# Autodesk Inventor assembly: ПД Модуль 200х140х75
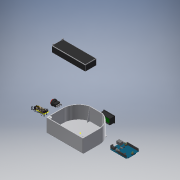
[picture p0: Inventor's stored thumbnail of the model, 180x180]
Saved by Autodesk Inventor 2019 (Build 230136000, 136)
## iProperties
Created: 2020-05-19
Part Number: ПД Модуль 200х140х75
Material: Типовые
Document SubType Name: Assembly
Designer: Surflay
Author: Surflay
## Documents named in this file (9)
- C:\Users\bossl\Desktop\Модуль ДУ Inventor\Дистанционная связь (модуль)\ПД Модуль 160х140х75.iam
- C:\Users\bossl\Desktop\Модуль ДУ Inventor\Дистанционная связь (модуль)\ПД Коробка 160х140х75.ipt
- C:\Users\bossl\Desktop\Модуль ДУ Inventor\Дистанционная связь (модуль)\РадиоМодуль.ipt
- C:\Users\bossl\Desktop\Модуль ДУ Inventor\Дистанционная связь (модуль)\Arduino UNO.ipt
- C:\Users\bossl\Desktop\Модуль ДУ Inventor\Дистанционная связь (модуль)\Аккумулятор.ipt
- C:\Users\bossl\Desktop\Модуль ДУ Inventor\Дистанционная связь (модуль)\Кнопка.ipt
- C:\Users\bossl\Desktop\Модуль ДУ Inventor\Дистанционная связь (модуль)\ВольтметрЦифровой.ipt
- C:\Users\bossl\Desktop\Модуль ДУ Inventor\Дистанционная связь (модуль)\NextionDisplay.ipt
- C:\Users\bossl\Desktop\Модуль ДУ Inventor\Дистанционная связь (модуль)\Джойстик.ipt
## Components (9 placed, 8 different names)
1. ПД Коробка 160х140х75:1
2. РадиоМодуль:1
3. Arduino UNO:1
4. Аккумулятор:1
5. Кнопка:1
6. ВольтметрЦифровой:1
7. NextionDisplay:1
8. Джойстик:1
9. Джойстик:2
## Component patterns: (2 elements, first: Джойстик:1)
